# Autodesk Inventor assembly: Cornerassembly_MIR
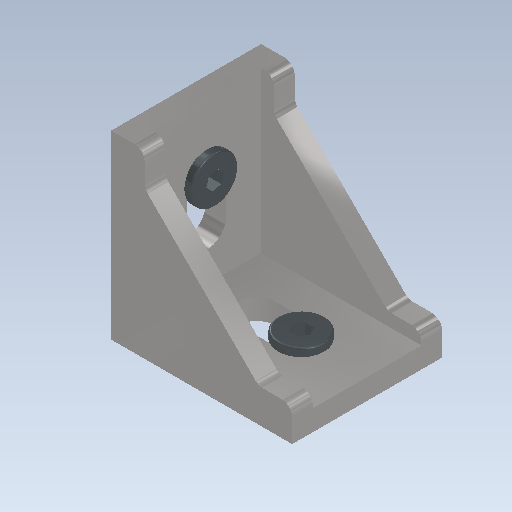
[picture p0: Inventor's stored thumbnail of the model, 512x512]
Saved by Autodesk Inventor 2020.2 (Build 242310000, 310)
## iProperties
Created: 2020-07-25
Part Number: Cornerassembly_MIR
Document SubType Name: Assembly
Designer: JK
Author: JK
## Documents named in this file (4)
- C:\Users\JK\Documents\Inventor\Mesa\Cornerassembly_MIR.iam
- C:\Users\JK\Documents\Inventor\Mesa\3030cornerbracket_MIR.ipt
- C:\Users\JK\Documents\Inventor\Mesa\T_Slot_Nut_Dropin_3030m5ipt_MIR1.ipt
- C:\Users\JK\Documents\Inventor\Mesa\M5x12BoltFlatHead_MIR.ipt
## Components (5 placed, 3 different names)
1. 3030cornerbracket_MIR:1 — Angle:2, Mate:6, Angle:1, Mate:3, Mate:8, Mate:7, Mate:5, Mate:4
2. T_Slot_Nut_Dropin_3030m5ipt_MIR1:1 — Angle:2, Mate:6, Mate:1
3. T_Slot_Nut_Dropin_3030m5ipt_MIR1:2 — Angle:1, Mate:3, Mate:2
4. M5x12BoltFlatHead_MIR:1 — Mate:8, Mate:7, Mate:1
5. M5x12BoltFlatHead_MIR:2 — Mate:5, Mate:4, Mate:2
## Relationships (10: Mate 8, Angle 2)
- Angle:2 (0 deg): 3030cornerbracket_MIR:1 ↔ T_Slot_Nut_Dropin_3030m5ipt_MIR1:1
- Mate:6: 3030cornerbracket_MIR:1 ↔ T_Slot_Nut_Dropin_3030m5ipt_MIR1:1
- Angle:1 (0 deg): 3030cornerbracket_MIR:1 ↔ T_Slot_Nut_Dropin_3030m5ipt_MIR1:2
- Mate:3: 3030cornerbracket_MIR:1 ↔ T_Slot_Nut_Dropin_3030m5ipt_MIR1:2
- Mate:8: 3030cornerbracket_MIR:1 ↔ M5x12BoltFlatHead_MIR:1
- Mate:7: 3030cornerbracket_MIR:1 ↔ M5x12BoltFlatHead_MIR:1
- Mate:1: T_Slot_Nut_Dropin_3030m5ipt_MIR1:1 ↔ M5x12BoltFlatHead_MIR:1
- Mate:5: 3030cornerbracket_MIR:1 ↔ M5x12BoltFlatHead_MIR:2
- Mate:4: 3030cornerbracket_MIR:1 ↔ M5x12BoltFlatHead_MIR:2
- Mate:2: T_Slot_Nut_Dropin_3030m5ipt_MIR1:2 ↔ M5x12BoltFlatHead_MIR:2
